# Autodesk Inventor assembly: Enclosure
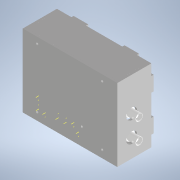
[picture p0: Inventor's stored thumbnail of the model, 180x180]
Saved by Autodesk Inventor 2020.3 (Build 243373000, 373)
## iProperties
Created: 2020-08-22
Part Number: Enclosure
Document SubType Name: Assembly
Designer: Scott Hanson
Author: Scott Hanson
## Documents named in this file (6)
- C:\Users\User\Documents\GitHub\BenchSignalGenerator\BenchSignalEnclosure\Enclosure.iam
- C:\Users\User\Documents\GitHub\BenchSignalGenerator\BenchSignalEnclosure\Base.ipt
- C:\Users\User\Documents\GitHub\BenchSignalGenerator\BenchSignalEnclosure\BenchSignalGenerator.ipt
- C:\Users\User\Documents\GitHub\BenchSignalGenerator\BenchSignalEnclosure\LongSide.ipt
- C:\Users\User\Documents\GitHub\BenchSignalGenerator\BenchSignalEnclosure\ShortSide.ipt
- C:\Users\User\Documents\GitHub\BenchSignalGenerator\BenchSignalEnclosure\ShortSideFront.ipt
## Components (6 placed, 5 different names)
1. Base:1 — Rotational:1, Rotational:2, Planar:1, Rotational:3, Rotational:4, Planar:2, Rotational:5, Planar:3, Rotational:6, Planar:4
2. BenchSignalGenerator:1 — Rotational:1, Rotational:2
3. LongSide:2 — Rotational:4, Planar:2
4. LongSide:3 — Planar:1, Rotational:3
5. ShortSide:1 — Rotational:5, Planar:3
6. ShortSideFront:1 — Rotational:6, Planar:4
## Relationships (10: RevoluteJoint 6, PlanarJoint 4)
- Rotational:1 [RevoluteJoint] (-10 mm): Base:1 ↔ BenchSignalGenerator:1
- Rotational:2 [RevoluteJoint] (-10 mm): Base:1 ↔ BenchSignalGenerator:1
- Planar:1: Base:1 ↔ LongSide:3
- Rotational:3 [RevoluteJoint]: Base:1 ↔ LongSide:3
- Rotational:4 [RevoluteJoint]: Base:1 ↔ LongSide:2
- Planar:2: Base:1 ↔ LongSide:2
- Rotational:5 [RevoluteJoint]: Base:1 ↔ ShortSide:1
- Planar:3: Base:1 ↔ ShortSide:1
- Rotational:6 [RevoluteJoint]: Base:1 ↔ ShortSideFront:1
- Planar:4: Base:1 ↔ ShortSideFront:1
